# Autodesk Inventor assembly: ダンパーアセンブリ
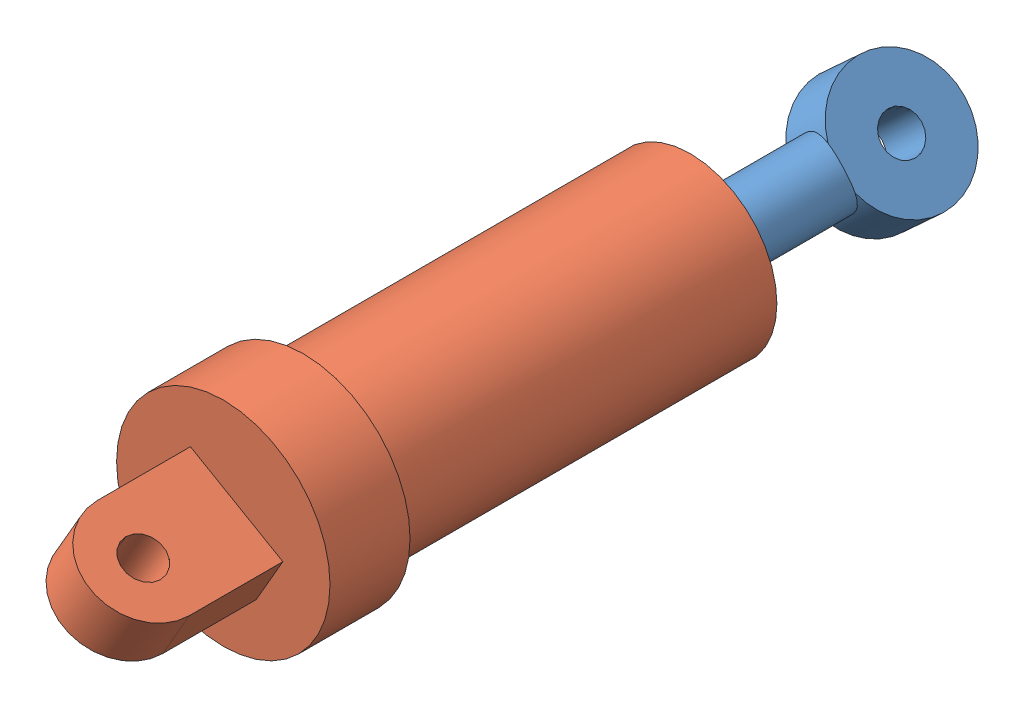
[picture p0: shaded view drawn from the part files that the assembly names]
Saved by Autodesk Inventor 2020.2 (Build 242310000, 310)
## iProperties
Created: 2018-03-29
Part Number: ダンパーアセンブリ
Material: 一般
Document SubType Name: Assembly
Designer: Takumi
Mass: 15 g
Surface Area: 26.818 cm^2
Volume: 4.2661 cm^3
Density: 3.51609 g/cm^3
Author: Takumi
## Documents named in this file (3)
- C:\Users\mozar\Desktop\院2年機\既製品\ダンパーアセンブリ.iam
- C:\Users\mozar\Desktop\院2年機\既製品\ダンパー下パーツ.ipt
- C:\Users\mozar\Desktop\院2年機\既製品\ダンパー上パーツ.ipt
## Components (2 placed, 2 different names)
1. ダンパー下パーツ:1 — メイト:1
2. ダンパー上パーツ:1 — メイト:1
## Relationships (1: Mate 1)
- メイト:1 [Mate]: ダンパー下パーツ:1 ↔ ダンパー上パーツ:1
